# Autodesk Inventor assembly: Gripper Assembly
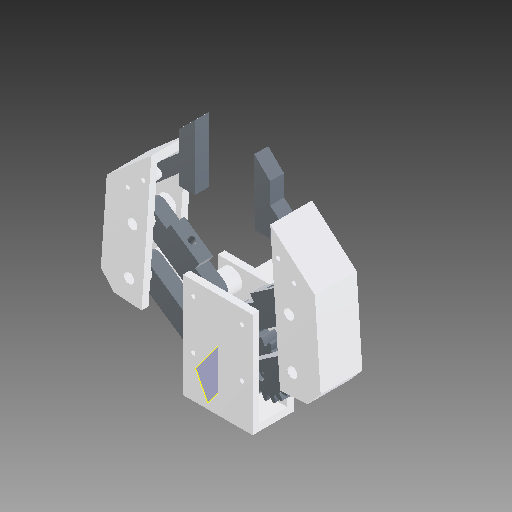
[picture p0: Inventor's stored thumbnail of the model, 512x512]
Saved by Autodesk Inventor 2017 (Build 210142000, 142)
## iProperties
Created: 2017-06-19
Part Number: Gripper Assembly
Document SubType Name: Assembly
Designer: Zach
Author: Zach
## Documents named in this file (12)
- C:\Users\zallen\Documents\GitHub\cr-laundry-robot\src\Body\Arm Assembly\Gripper Assembly\Gripper Assembly.iam
- C:\Users\zallen\Documents\GitHub\cr-laundry-robot\src\Body\Arm Assembly\Gripper Assembly\GA001.ipt
- C:\Users\zallen\Documents\GitHub\cr-laundry-robot\src\Body\Arm Assembly\Gripper Assembly\GA002.ipt
- C:\Users\zallen\Documents\GitHub\cr-laundry-robot\src\Body\Arm Assembly\Gripper Assembly\GA003.ipt
- C:\Users\zallen\Documents\GitHub\cr-laundry-robot\src\Body\Arm Assembly\Gripper Assembly\GA004.ipt
- C:\Users\zallen\Documents\GitHub\cr-laundry-robot\src\Body\Arm Assembly\Gripper Assembly\GA005.ipt
- C:\Users\zallen\Documents\GitHub\cr-laundry-robot\src\Body\Arm Assembly\Gripper Assembly\GA006.ipt
- C:\Users\zallen\Documents\GitHub\cr-laundry-robot\src\Body\Arm Assembly\Gripper Assembly\GA007.ipt
- C:\Users\zallen\Documents\GitHub\cr-laundry-robot\src\Body\Arm Assembly\Gripper Assembly\GA008.ipt
- C:\Users\zallen\Documents\GitHub\cr-laundry-robot\src\Body\Arm Assembly\Gripper Assembly\GA009.ipt
- C:\Users\zallen\Documents\GitHub\cr-laundry-robot\lib\Futaba S3114\FutabaS3114.ipt
- C:\Users\zallen\Documents\GitHub\cr-laundry-robot\src\Body\Arm Assembly\Gripper Assembly\GA010.ipt
## Components (15 placed, 11 different names)
1. GA001:1 — Mate:1, Mate:5, Mate:7, Mate:9, Mate:12, Mate:16, Mate:20, Mate:21, Mate:22, Mate:33, Mate:38, Mate:39, Mate:40, Mate:42, Mate:44, Mate:45, Mate:46, Mate:48, Mate:49, Mate:50, Mate:51, Mate:52, Mate:53
2. GA002:1 — Mate:1, Mate:10, Mate:11, Mate:33, Rotation:1
3. GA003:1 — Mate:5, Mate:16, Mate:18
4. GA003:2 — Mate:7, Mate:23, Mate:41
5. GA004:1 — Mate:9, Mate:10, Mate:11, Mate:17, Mate:34, Symmetry:1
6. GA004:2 — Mate:12, Mate:24, Mate:35, Symmetry:1, Mate:47
7. GA005:1 — Mate:17, Mate:18, Mate:29, Mate:30, Mate:34, Mate:37, Symmetry:2
8. GA005:2 — Mate:23, Mate:24, Mate:26, Mate:27, Mate:35, Mate:36, Mate:41, Symmetry:2
9. GA006:1 — Mate:20, Mate:21, Mate:22
10. GA007:1 — Mate:26, Mate:27, Mate:36
11. GA007:2 — Mate:29, Mate:30, Mate:37
12. GA008:1 — Mate:42, Mate:44, Mate:47
13. GA009:1 — Mate:45, Mate:46, Rotation:1
14. FutabaS3114:1 — Mate:48, Mate:49, Mate:50
15. GA010:1 — Mate:51, Mate:52, Mate:53
## Relationships (42: Mate 39, Symmetry 2, RelateRotation 1)
- Mate:1: GA001:1 ↔ GA002:1
- Mate:5: GA001:1 ↔ GA003:1
- Mate:7: GA001:1 ↔ GA003:2
- Mate:9: GA001:1 ↔ GA004:1
- Mate:10: GA002:1 ↔ GA004:1
- Mate:11: GA002:1 ↔ GA004:1
- Mate:12: GA001:1 ↔ GA004:2
- Mate:16: GA001:1 ↔ GA003:1
- Mate:17: GA004:1 ↔ GA005:1
- Mate:18: GA003:1 ↔ GA005:1
- Mate:20: GA001:1 ↔ GA006:1
- Mate:21: GA001:1 ↔ GA006:1
- Mate:22: GA001:1 ↔ GA006:1
- Mate:23: GA003:2 ↔ GA005:2
- Mate:24: GA004:2 ↔ GA005:2
- Mate:26: GA005:2 ↔ GA007:1
- Mate:27: GA005:2 ↔ GA007:1
- Mate:29: GA005:1 ↔ GA007:2
- Mate:30: GA005:1 ↔ GA007:2
- Mate:33: GA001:1 ↔ GA002:1
- Mate:34: GA004:1 ↔ GA005:1
- Mate:35: GA004:2 ↔ GA005:2
- Mate:36: GA005:2 ↔ GA007:1
- Mate:37: GA005:1 ↔ GA007:2
- Mate:38: GA001:1
- Mate:39: GA001:1
- Mate:40: GA001:1
- Symmetry:1: GA004:1 ↔ GA004:2
- Mate:41: GA003:2 ↔ GA005:2
- Symmetry:2: GA005:1 ↔ GA005:2
- Mate:42: GA001:1 ↔ GA008:1
- Mate:44: GA001:1 ↔ GA008:1
- Mate:45: GA001:1 ↔ GA009:1
- Mate:46: GA001:1 ↔ GA009:1
- Rotation:1 [RelateRotation] (0.5 ul): GA002:1 ↔ GA009:1
- Mate:47: GA004:2 ↔ GA008:1
- Mate:48: GA001:1 ↔ FutabaS3114:1
- Mate:49: GA001:1 ↔ FutabaS3114:1
- Mate:50: GA001:1 ↔ FutabaS3114:1
- Mate:51: GA001:1 ↔ GA010:1
- Mate:52: GA001:1 ↔ GA010:1
- Mate:53: GA001:1 ↔ GA010:1
